# Autodesk Inventor assembly: ConveyorBaseAssembly
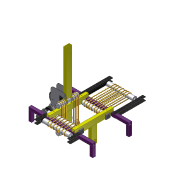
[picture p0: Inventor's stored thumbnail of the model, 180x180]
Saved by Autodesk Inventor 2012 (Build 160160000, 160)
## iProperties
Created: 2012-01-21
Part Number: ConveyorBaseAssembly
Document SubType Name: Assembly
Designer: JesseK
Mass: 3887.87 g
Surface Area: 12449.6 cm^2
Volume: 2367.1 cm^3
Density: 1.64246 g/cm^3
Author: JesseK
## Documents named in this file (20)
- Z:\UserData\Documents\Inventor\team1885frc\Robot2012\ConveyorBaseAssembly.iam
- Z:\UserData\Documents\Inventor\team1885frc\Robot2012\Drawings\ConveyorDriveSide_20Jan.iam
- Z:\UserData\Documents\Inventor\team1885frc\Robot2012\Drawings\ConveyorIdleSide_20Jan.iam
- Z:\UserData\Documents\Inventor\team1885frc\Robot2012\Drawings\ConveyorCrossFrame_20Jan.iam
- Z:\UserData\Documents\Inventor\team1885frc\Robot2012\Conveyor2\Conveyor_Roller_Cross.ipt
- Z:\UserData\Documents\Inventor\team1885frc\Robot2012\ConveyorBase\Roller_VerticalConveyor_Middle.ipt
- Z:\UserData\Documents\Inventor\team1885frc\Robot2012\ConveyorBase\Roller_VerticalConveyor_Outer.ipt
- Z:\UserData\Documents\Inventor\team1885frc\Robot2012\ConveyorBase\Belt_VerticalConveyor_Outer.ipt
- Z:\UserData\Documents\Inventor\team1885frc\Robot2012\Conveyor3\Frame_OuterConveyorMount_Front.ipt
- Z:\UserData\Documents\Inventor\team1885frc\Robot2012\Conveyor3\Frame_OuterConveyorMount_Rear.ipt
- Z:\UserData\Documents\Inventor\team1885frc\Robot2012\Conveyor2\Conveyor_Roller_Outer.ipt
- Z:\UserData\Documents\Inventor\team1885frc\Robot2012\ConveyorBase\Belt_HorizontalIntake_Front.ipt
- Z:\UserData\Documents\Inventor\team1885frc\Robot2012\ConveyorBase\Belt_HorizontalIntake_Rear.ipt
- Z:\UserData\Documents\Inventor\team1885frc\Robot2012\Misc\Generic_Pillow_Block.iam
- Z:\UserData\Documents\Inventor\team1885frc\Robot2012\Conveyor3\Plate_VerticalConveyorMotorMount.ipt
- Z:\UserData\Documents\Inventor\team1885frc\IFI\Imported Components\IFI-WHEEL-ASSY-410-38\IFI-WHEEL-ASSY-410-38.iam
- Z:\UserData\Documents\Inventor\team1885frc\AndyMark\CIMpleBox\CIMpleBoxStandalone.iam
- Z:\UserData\Documents\Inventor\team1885frc\AndyMark\AMPlanetary2\AMPlanetary2.iam
- Z:\UserData\Documents\Inventor\team1885frc\Banebots\BaneBots_RS-550.ipt
- Z:\UserData\Documents\Inventor\team1885frc\Robot2012\Conveyor2\Conveyor_Roller_MainOuter.ipt
## Components (50 placed, 19 different names)
1. ConveyorDriveSide_20Jan:1 [sub-assembly] — Mate:2, Flush:1, Mate:6, Mate:7, Mate:11, Mate:12, Mate:13, Mate:14, Mate:15, Mate:55, Mate:56, Mate:57, Mate:60, Mate:66, Mate:67, Mate:68, Mate:69, Mate:72, Mate:73, Mate:74, Mate:75, Mate:76
2. ConveyorIdleSide_20Jan:1 [sub-assembly] — Mate:1, Mate:3, Mate:8, Mate:9, Flush:27, Mate:55, Mate:63, Mate:64, Mate:65, Mate:70, Mate:71
3. ConveyorCrossFrame_20Jan:1 [sub-assembly] — Mate:1, Mate:2, Mate:3, Flush:1, Flush:2, Mate:30, Mate:56, Mate:58, Mate:59
4. ConveyorCrossFrame_20Jan:2 [sub-assembly] — Mate:6, Flush:2, Mate:7, Mate:32, Mate:34, Mate:35, Mate:61, Mate:62
5. Conveyor_Roller_Cross:1 — Mate:8, Flush:3, Mate:40, Tangent:12, Tangent:13, Tangent:14, Tangent:15, Tangent:16, Tangent:17
6. Conveyor_Roller_Cross:2 — Mate:9, Flush:3, Tangent:18, Tangent:19, Tangent:20, Tangent:21, Tangent:22, Tangent:23, Tangent:24, Tangent:25
7. Roller_VerticalConveyor_Middle:1 — Mate:72
8. Roller_VerticalConveyor_Middle:2 — Mate:11
9. Roller_VerticalConveyor_Outer:1 — Mate:15, Flush:4, Tangent:3, Tangent:4, Tangent:5
10. Roller_VerticalConveyor_Outer:2 — Mate:14, Flush:5, Tangent:1, Tangent:6, Tangent:7, Tangent:8
11. Roller_VerticalConveyor_Outer:3 — Mate:13, Flush:5, Mate:16, Mate:21, Mate:23
12. Roller_VerticalConveyor_Outer:4 — Mate:12, Flush:4, Mate:17, Mate:18, Mate:19
13. Belt_VerticalConveyor_Outer:1 — Mate:16, Tangent:1, Tangent:6
14. Belt_VerticalConveyor_Outer:2 — Mate:17, Tangent:3
15. Belt_VerticalConveyor_Outer:3 — Mate:21, Tangent:7
16. Belt_VerticalConveyor_Outer:5 — Mate:23, Tangent:8
17. Belt_VerticalConveyor_Outer:6 — Mate:18, Tangent:5
18. Belt_VerticalConveyor_Outer:7 — Mate:19, Tangent:4
19. Frame_OuterConveyorMount_Front:1 — Flush:27, Mate:28, Mate:30, Mate:38
20. Frame_OuterConveyorMount_Rear:1 — Mate:32, Mate:34, Mate:37, Mate:39, Mate:60, Mate:61
21. Frame_OuterConveyorMount_Front:2 — Mate:28, Mate:57, Mate:58, Mate:59
22. Frame_OuterConveyorMount_Rear:2 — Mate:35, Mate:37, Mate:62, Mate:63
23. Conveyor_Roller_Outer:1 — Mate:39, Flush:6, Mate:48, Mate:49, Mate:50, Mate:51, Mate:52, Mate:53, Mate:54
24. Conveyor_Roller_Outer:2 — Mate:38, Flush:6, Tangent:10, Mate:41, Mate:42, Mate:43, Mate:44, Mate:45, Mate:47
25. Belt_HorizontalIntake_Front:1 — Mate:40, Tangent:10
26. Belt_HorizontalIntake_Front:2 — Mate:41, Tangent:16
27. Belt_HorizontalIntake_Front:3 — Mate:42, Tangent:15
28. Belt_HorizontalIntake_Front:4 — Mate:43, Tangent:14
29. Belt_HorizontalIntake_Front:5 — Mate:44, Tangent:12
30. Belt_HorizontalIntake_Front:6 — Mate:45, Tangent:17
31. Belt_HorizontalIntake_Front:8 — Mate:47, Tangent:13
32. Belt_HorizontalIntake_Rear:1 — Mate:48, Tangent:18, Tangent:25
33. Belt_HorizontalIntake_Rear:2 — Mate:54, Tangent:23
34. Belt_HorizontalIntake_Rear:3 — Mate:53, Tangent:22
35. Belt_HorizontalIntake_Rear:4 — Mate:52, Tangent:21
36. Belt_HorizontalIntake_Rear:5 — Mate:51, Tangent:20
37. Belt_HorizontalIntake_Rear:6 — Mate:50, Tangent:24
38. Belt_HorizontalIntake_Rear:7 — Mate:49, Tangent:19
39. Generic_Pillow_Block:1 [sub-assembly] — Mate:65, Mate:71
40. Generic_Pillow_Block:2 [sub-assembly] — Mate:64, Mate:70
41. Generic_Pillow_Block:3 [sub-assembly] — Mate:67, Mate:68, Mate:87
42. Generic_Pillow_Block:4 [sub-assembly] — Mate:66, Mate:69, Mate:86, Mate:88
43. Plate_VerticalConveyorMotorMount:1 — Mate:73, Mate:75, Mate:85
44. Plate_VerticalConveyorMotorMount:2 — Mate:74, Mate:76, Mate:78, Mate:79, Mate:80, Mate:85
45. IFI-WHEEL-ASSY-410-38:1 [sub-assembly] — Mate:78
46. CIMpleBoxStandalone:1 [sub-assembly] — Mate:79, Mate:80, Mate:82, Mate:89
47. AMPlanetary2:1 [sub-assembly] — Mate:82, Mate:83, Mate:84, Mate:89
48. BaneBots_RS-550:1 — Mate:83, Mate:84
49. Conveyor_Roller_MainOuter:1 — Mate:87, Flush:28
50. Conveyor_Roller_MainOuter:2 — Mate:86, Flush:28, Mate:88
## Relationships (103: Mate 73, Tangent 22, Flush 8)
- Mate:1: ConveyorIdleSide_20Jan:1 ↔ ConveyorCrossFrame_20Jan:1
- Mate:2: ConveyorDriveSide_20Jan:1 ↔ ConveyorCrossFrame_20Jan:1
- Mate:3: ConveyorIdleSide_20Jan:1 ↔ ConveyorCrossFrame_20Jan:1
- Flush:1: ConveyorDriveSide_20Jan:1 ↔ ConveyorCrossFrame_20Jan:1
- Mate:6: ConveyorDriveSide_20Jan:1 ↔ ConveyorCrossFrame_20Jan:2
- Flush:2: ConveyorCrossFrame_20Jan:1 ↔ ConveyorCrossFrame_20Jan:2
- Mate:7: ConveyorDriveSide_20Jan:1 ↔ ConveyorCrossFrame_20Jan:2
- Mate:8: ConveyorIdleSide_20Jan:1 ↔ Conveyor_Roller_Cross:1
- Mate:9: ConveyorIdleSide_20Jan:1 ↔ Conveyor_Roller_Cross:2
- Flush:3: Conveyor_Roller_Cross:1 ↔ Conveyor_Roller_Cross:2
- Mate:11: ConveyorDriveSide_20Jan:1 ↔ Roller_VerticalConveyor_Middle:2
- Mate:12: ConveyorDriveSide_20Jan:1 ↔ Roller_VerticalConveyor_Outer:4
- Mate:13: ConveyorDriveSide_20Jan:1 ↔ Roller_VerticalConveyor_Outer:3
- Mate:14: ConveyorDriveSide_20Jan:1 ↔ Roller_VerticalConveyor_Outer:2
- Mate:15: ConveyorDriveSide_20Jan:1 ↔ Roller_VerticalConveyor_Outer:1
- Flush:4: Roller_VerticalConveyor_Outer:1 ↔ Roller_VerticalConveyor_Outer:4
- Flush:5: Roller_VerticalConveyor_Outer:2 ↔ Roller_VerticalConveyor_Outer:3
- Mate:16: Roller_VerticalConveyor_Outer:3 ↔ Belt_VerticalConveyor_Outer:1
- Tangent:1: Roller_VerticalConveyor_Outer:2 ↔ Belt_VerticalConveyor_Outer:1
- Mate:17: Roller_VerticalConveyor_Outer:4 ↔ Belt_VerticalConveyor_Outer:2
- Mate:18: Roller_VerticalConveyor_Outer:4 ↔ Belt_VerticalConveyor_Outer:6
- Mate:19: Roller_VerticalConveyor_Outer:4 ↔ Belt_VerticalConveyor_Outer:7
- Mate:21: Roller_VerticalConveyor_Outer:3 ↔ Belt_VerticalConveyor_Outer:3
- Mate:23: Roller_VerticalConveyor_Outer:3 ↔ Belt_VerticalConveyor_Outer:5
- Tangent:3: Roller_VerticalConveyor_Outer:1 ↔ Belt_VerticalConveyor_Outer:2
- Tangent:4: Roller_VerticalConveyor_Outer:1 ↔ Belt_VerticalConveyor_Outer:7
- Tangent:5: Roller_VerticalConveyor_Outer:1 ↔ Belt_VerticalConveyor_Outer:6
- Tangent:6: Roller_VerticalConveyor_Outer:2 ↔ Belt_VerticalConveyor_Outer:1
- Tangent:7: Roller_VerticalConveyor_Outer:2 ↔ Belt_VerticalConveyor_Outer:3
- Tangent:8: Roller_VerticalConveyor_Outer:2 ↔ Belt_VerticalConveyor_Outer:5
- Flush:27 (-31.75 mm): ConveyorIdleSide_20Jan:1 ↔ Frame_OuterConveyorMount_Front:1
- Mate:28: Frame_OuterConveyorMount_Front:1 ↔ Frame_OuterConveyorMount_Front:2
- Mate:30: ConveyorCrossFrame_20Jan:1 ↔ Frame_OuterConveyorMount_Front:1
- Mate:32: ConveyorCrossFrame_20Jan:2 ↔ Frame_OuterConveyorMount_Rear:1
- Mate:34: ConveyorCrossFrame_20Jan:2 ↔ Frame_OuterConveyorMount_Rear:1
- Mate:35: ConveyorCrossFrame_20Jan:2 ↔ Frame_OuterConveyorMount_Rear:2
- Mate:37: Frame_OuterConveyorMount_Rear:1 ↔ Frame_OuterConveyorMount_Rear:2
- Mate:38: Frame_OuterConveyorMount_Front:1 ↔ Conveyor_Roller_Outer:2
- Mate:39: Frame_OuterConveyorMount_Rear:1 ↔ Conveyor_Roller_Outer:1
- Flush:6: Conveyor_Roller_Outer:1 ↔ Conveyor_Roller_Outer:2
- Mate:40: Conveyor_Roller_Cross:1 ↔ Belt_HorizontalIntake_Front:1
- Tangent:10: Conveyor_Roller_Outer:2 ↔ Belt_HorizontalIntake_Front:1
- Mate:41: Conveyor_Roller_Outer:2 ↔ Belt_HorizontalIntake_Front:2
- Mate:42: Conveyor_Roller_Outer:2 ↔ Belt_HorizontalIntake_Front:3
- Mate:43: Conveyor_Roller_Outer:2 ↔ Belt_HorizontalIntake_Front:4
- Mate:44: Conveyor_Roller_Outer:2 ↔ Belt_HorizontalIntake_Front:5
- Mate:45: Conveyor_Roller_Outer:2 ↔ Belt_HorizontalIntake_Front:6
- Mate:47: Conveyor_Roller_Outer:2 ↔ Belt_HorizontalIntake_Front:8
- Tangent:12: Conveyor_Roller_Cross:1 ↔ Belt_HorizontalIntake_Front:5
- Tangent:13: Conveyor_Roller_Cross:1 ↔ Belt_HorizontalIntake_Front:8
- Tangent:14: Conveyor_Roller_Cross:1 ↔ Belt_HorizontalIntake_Front:4
- Tangent:15: Conveyor_Roller_Cross:1 ↔ Belt_HorizontalIntake_Front:3
- Tangent:16: Conveyor_Roller_Cross:1 ↔ Belt_HorizontalIntake_Front:2
- Tangent:17: Conveyor_Roller_Cross:1 ↔ Belt_HorizontalIntake_Front:6
- Mate:48: Conveyor_Roller_Outer:1 ↔ Belt_HorizontalIntake_Rear:1
- Tangent:18: Conveyor_Roller_Cross:2 ↔ Belt_HorizontalIntake_Rear:1
- Mate:49: Conveyor_Roller_Outer:1 ↔ Belt_HorizontalIntake_Rear:7
- Mate:50: Conveyor_Roller_Outer:1 ↔ Belt_HorizontalIntake_Rear:6
- Mate:51: Conveyor_Roller_Outer:1 ↔ Belt_HorizontalIntake_Rear:5
- Mate:52: Conveyor_Roller_Outer:1 ↔ Belt_HorizontalIntake_Rear:4
- Mate:53: Conveyor_Roller_Outer:1 ↔ Belt_HorizontalIntake_Rear:3
- Mate:54: Conveyor_Roller_Outer:1 ↔ Belt_HorizontalIntake_Rear:2
- Tangent:19: Conveyor_Roller_Cross:2 ↔ Belt_HorizontalIntake_Rear:7
- Tangent:20: Conveyor_Roller_Cross:2 ↔ Belt_HorizontalIntake_Rear:5
- Tangent:21: Conveyor_Roller_Cross:2 ↔ Belt_HorizontalIntake_Rear:4
- Tangent:22: Conveyor_Roller_Cross:2 ↔ Belt_HorizontalIntake_Rear:3
- Tangent:23: Conveyor_Roller_Cross:2 ↔ Belt_HorizontalIntake_Rear:2
- Tangent:24: Conveyor_Roller_Cross:2 ↔ Belt_HorizontalIntake_Rear:6
- Tangent:25: Conveyor_Roller_Cross:2 ↔ Belt_HorizontalIntake_Rear:1
- Mate:55 (203.2 mm): ConveyorDriveSide_20Jan:1 ↔ ConveyorIdleSide_20Jan:1
- Mate:56 (-165.1 mm): ConveyorDriveSide_20Jan:1 ↔ ConveyorCrossFrame_20Jan:1
- Mate:57 (6.35 mm): ConveyorDriveSide_20Jan:1 ↔ Frame_OuterConveyorMount_Front:2
- Mate:58: ConveyorCrossFrame_20Jan:1 ↔ Frame_OuterConveyorMount_Front:2
- Mate:59: ConveyorCrossFrame_20Jan:1 ↔ Frame_OuterConveyorMount_Front:2
- Mate:60 (6.35 mm): ConveyorDriveSide_20Jan:1 ↔ Frame_OuterConveyorMount_Rear:1
- Mate:61: ConveyorCrossFrame_20Jan:2 ↔ Frame_OuterConveyorMount_Rear:1
- Mate:62: ConveyorCrossFrame_20Jan:2 ↔ Frame_OuterConveyorMount_Rear:2
- Mate:63 (6.35 mm): ConveyorIdleSide_20Jan:1 ↔ Frame_OuterConveyorMount_Rear:2
- Mate:64: ConveyorIdleSide_20Jan:1 ↔ Generic_Pillow_Block:2
- Mate:65: ConveyorIdleSide_20Jan:1 ↔ Generic_Pillow_Block:1
- Mate:66: ConveyorDriveSide_20Jan:1 ↔ Generic_Pillow_Block:4
- Mate:67: ConveyorDriveSide_20Jan:1 ↔ Generic_Pillow_Block:3
- Mate:68: ConveyorDriveSide_20Jan:1 ↔ Generic_Pillow_Block:3
- Mate:69: ConveyorDriveSide_20Jan:1 ↔ Generic_Pillow_Block:4
- Mate:70: ConveyorIdleSide_20Jan:1 ↔ Generic_Pillow_Block:2
- Mate:71: ConveyorIdleSide_20Jan:1 ↔ Generic_Pillow_Block:1
- Mate:72: ConveyorDriveSide_20Jan:1 ↔ Roller_VerticalConveyor_Middle:1
- Mate:73: ConveyorDriveSide_20Jan:1 ↔ Plate_VerticalConveyorMotorMount:1
- Mate:74: ConveyorDriveSide_20Jan:1 ↔ Plate_VerticalConveyorMotorMount:2
- Mate:75: ConveyorDriveSide_20Jan:1 ↔ Plate_VerticalConveyorMotorMount:1
- Mate:76: ConveyorDriveSide_20Jan:1 ↔ Plate_VerticalConveyorMotorMount:2
- Mate:78: Plate_VerticalConveyorMotorMount:2 ↔ IFI-WHEEL-ASSY-410-38:1
- Mate:79: Plate_VerticalConveyorMotorMount:2 ↔ CIMpleBoxStandalone:1
- Mate:80: Plate_VerticalConveyorMotorMount:2 ↔ CIMpleBoxStandalone:1
- Mate:82: CIMpleBoxStandalone:1 ↔ AMPlanetary2:1
- Mate:83: AMPlanetary2:1 ↔ BaneBots_RS-550:1
- Mate:84: AMPlanetary2:1 ↔ BaneBots_RS-550:1
- Mate:85: Plate_VerticalConveyorMotorMount:1 ↔ Plate_VerticalConveyorMotorMount:2
- Mate:86: Generic_Pillow_Block:4 ↔ Conveyor_Roller_MainOuter:2
- Mate:87: Generic_Pillow_Block:3 ↔ Conveyor_Roller_MainOuter:1
- Flush:28: Conveyor_Roller_MainOuter:1 ↔ Conveyor_Roller_MainOuter:2
- Mate:88: Generic_Pillow_Block:4 ↔ Conveyor_Roller_MainOuter:2
- Mate:89: CIMpleBoxStandalone:1 ↔ AMPlanetary2:1
